# Autodesk Inventor assembly: fuse
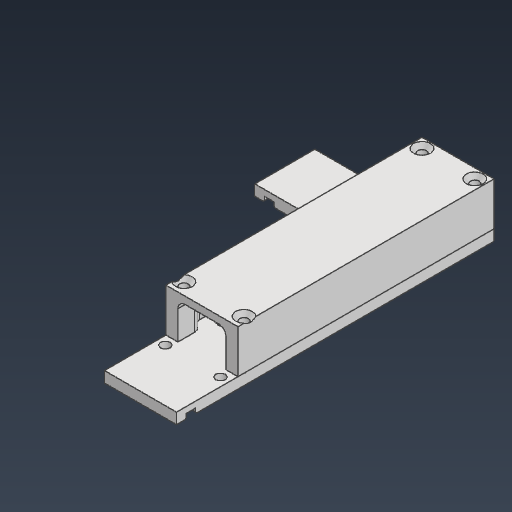
[picture p0: Inventor's stored thumbnail of the model, 512x512]
Saved by Autodesk Inventor 2023 (Build 270158000, 158)
## iProperties
Created: 2025-12-26
Part Number: fuse
Document SubType Name: Assembly
Designer: szymo
Author: szymo
## Documents named in this file (4)
- D:\tech\diy\e-skateboard\projekcik-inventor\fuse.iam
- D:\tech\diy\e-skateboard\projekcik-inventor\fusion_hold.ipt
- D:\tech\diy\e-skateboard\projekcik-inventor\fuse_holder_cover.ipt
- D:\tech\diy\e-skateboard\projekcik-inventor\Assembly - FUSE.iam
## Components (3 placed, 3 different names)
1. Assembly - FUSE:1 [sub-assembly]
2. fuse_holder_cover:1
3. fusion_hold:1
## Relationships (4: Flush 4)
- [Flush]: fuse_holder_cover:1 ↔ fusion_hold:1
- [Flush]: fuse_holder_cover:1 ↔ fusion_hold:1
- [Flush]: Assembly - FUSE:1 ↔ fusion_hold:1
- [Flush]: Assembly - FUSE:1 ↔ fusion_hold:1
## Named parameters: d2_d3 = 0 mm
